# Autodesk Inventor assembly: MONTAGEM_MANCAL
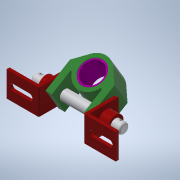
[picture p0: Inventor's stored thumbnail of the model, 180x180]
Saved by Autodesk Inventor 2020.4 (Build 244396000, 396)
## iProperties
Created: 2016-02-21
Part Number: MONTAGEM_MANCAL
Document SubType Name: Assembly
Designer: Everton
Author: Everton
## Documents named in this file (5)
- C:\Users\Alison\Documents\TCC\Desenhos e Montagem\desenhos e montagems inventor 15\MONTAGEM_MANCAL.iam
- C:\Users\Alison\Documents\TCC\Desenhos e Montagem\desenhos e montagems inventor 15\MANCAL_MOVEL.ipt
- C:\Users\Alison\Documents\TCC\Desenhos e Montagem\desenhos e montagems inventor 15\MANCAL_SUPORTE_EIXO.ipt
- C:\Users\Alison\Documents\TCC\Desenhos e Montagem\desenhos e montagems inventor 15\EIXO_16MM.ipt
- C:\Users\Alison\Documents\TCC\Desenhos e Montagem\desenhos e montagems inventor 15\BUCHA.ipt
## Components (5 placed, 4 different names)
1. MANCAL_MOVEL:1 — Mate:1, Mate:2, Angle:1
2. MANCAL_SUPORTE_EIXO:1 — Mate:1, Mate:2, Mate:3, Mate:4, Mate:8, Flush:2, Angle:1
3. MANCAL_MOVEL:2 — Mate:3, Mate:4, Mate:5
4. EIXO_16MM:1 — Mate:5
5. BUCHA:2 — Mate:8, Flush:2
## Relationships (8: Mate 6, Flush 1, Angle 1)
- Mate:1: MANCAL_MOVEL:1 ↔ MANCAL_SUPORTE_EIXO:1
- Mate:2 (0.2 mm): MANCAL_MOVEL:1 ↔ MANCAL_SUPORTE_EIXO:1
- Mate:3: MANCAL_SUPORTE_EIXO:1 ↔ MANCAL_MOVEL:2
- Mate:4: MANCAL_SUPORTE_EIXO:1 ↔ MANCAL_MOVEL:2
- Mate:5: MANCAL_MOVEL:2 ↔ EIXO_16MM:1
- Mate:8: MANCAL_SUPORTE_EIXO:1 ↔ BUCHA:2
- Flush:2: MANCAL_SUPORTE_EIXO:1 ↔ BUCHA:2
- Angle:1 (31 deg): MANCAL_MOVEL:1 ↔ MANCAL_SUPORTE_EIXO:1
